# Autodesk Inventor assembly: chamber_assembly_3Dprint
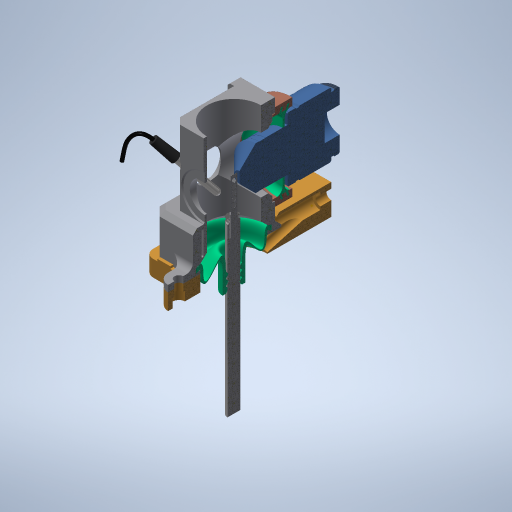
[picture p0: Inventor's stored thumbnail of the model, 512x512]
Saved by Autodesk Inventor 2023.3 (Build 273359000, 359)
## iProperties
Created: 2023-02-16
Part Number: chamber_assembly_3Dprint
Document SubType Name: Assembly
Designer: splath
Author: splath
## Documents named in this file (11)
- Z:\groups\stelzer-opticlab\CAD\mDSLM\New\chamber\chamber_assembly_3Dprint.iam
- Z:\groups\stelzer-opticlab\CAD\mDSLM\New\chamber\chamber_V2_new.ipt
- Z:\groups\stelzer-opticlab\CAD\mDSLM\New\chamber\objective_sealing\Sealingring_holder.ipt
- Z:\groups\stelzer-opticlab\CAD\mDSLM\New\chamber\bottom_rod_sealing\smooth_bellows\rod_seal_friction.ipt
- Z:\groups\stelzer-opticlab\CAD\mDSLM\New\chamber\objective_sealing\Sealingring.ipt
- Z:\groups\stelzer-opticlab\CAD\DSLM_accessories\specimen_holder\specimen_holder_rod_6mm.ipt
- Z:\groups\stelzer-opticlab\CAD\DSLM_accessories\specimen_holder\5_multi_beetle_holder.ipt
- Z:\groups\stelzer-opticlab\CAD\mDSLM\New\chamber\chamber bottom seal plate.ipt
- Z:\groups\stelzer-opticlab\CAD\mDSLM\New\TempSensor_RS-762-1134.ipt
- Z:\groups\stelzer-opticlab\CAD\mDSLM\New\chamber\bottom_rod_sealing\smooth_bellows\rod_seal_friction_folded.ipt
- Z:\groups\stelzer-opticlab\CAD\mDSLM\New\chamber\zeiss N-Achroplan 10x.ipt
## Components (10 placed, 10 different names)
1. chamber_V2_new:1 — Insert:1, Mate:1, Insert:2, Insert:3, Angle:1, Rigid:1, Mate:4, Mate:5
2. chamber bottom seal plate:1 — Mate:1, Insert:1
3. Sealingring_holder:1 — Insert:2, Insert:4
4. rod_seal_friction:1 — Insert:3, Mate:2, Rigid:2
5. Sealingring:1 — Insert:4
6. specimen_holder_rod_6mm:1 — Mate:2, Mate:3
7. 5_multi_beetle_holder:1 — Mate:3, Angle:1
8. TempSensor_RS-762-1134:1 — Rigid:1
9. rod_seal_friction_folded:1 — Rigid:2
10. zeiss N-Achroplan 10x:1 — Mate:4, Mate:5
## Relationships (12: Mate 5, Insert 4, WeldJoint 2, Angle 1)
- Insert:1: chamber_V2_new:1 ↔ chamber bottom seal plate:1
- Mate:1: chamber_V2_new:1 ↔ chamber bottom seal plate:1
- Insert:2: chamber_V2_new:1 ↔ Sealingring_holder:1
- Insert:3: chamber_V2_new:1 ↔ rod_seal_friction:1
- Insert:4: Sealingring_holder:1 ↔ Sealingring:1
- Mate:2: rod_seal_friction:1 ↔ specimen_holder_rod_6mm:1
- Mate:3: specimen_holder_rod_6mm:1 ↔ 5_multi_beetle_holder:1
- Angle:1 (0 deg): chamber_V2_new:1 ↔ 5_multi_beetle_holder:1
- Rigid:1 [WeldJoint] (2 mm): chamber_V2_new:1 ↔ TempSensor_RS-762-1134:1
- Rigid:2 [WeldJoint]: rod_seal_friction:1 ↔ rod_seal_friction_folded:1
- Mate:4: chamber_V2_new:1 ↔ zeiss N-Achroplan 10x:1
- Mate:5 (2.7 mm): chamber_V2_new:1 ↔ zeiss N-Achroplan 10x:1
## Named parameters: Sealing_offset = 0 mm
